# Autodesk Inventor assembly: TopOfRobot
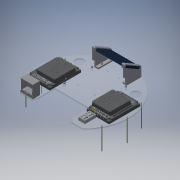
[picture p0: Inventor's stored thumbnail of the model, 180x180]
Saved by Autodesk Inventor 2019 (Build 230136000, 136)
## iProperties
Created: 2019-10-01
Part Number: TopOfRobot
Document SubType Name: Assembly
Designer: james
Author: james
## Documents named in this file (10)
- F:\JimsDesign\Jims2020FTC\TopOfRobot.iam
- F:\JimsDesign\Jims2020FTC\TopPlate.ipt
- F:\JimsDesign\Library\RevRobotics\REV-31-1153.ipt
- F:\JimsDesign\Jims2020FTC\CameraMount v4.ipt
- F:\JimsDesign\Jims2020FTC\SidePeg.ipt
- F:\JimsDesign\Jims2020FTC\CurrentMonitorBlock.ipt
- F:\JimsDesign\Jims2020FTC\PhoneStandLeft.ipt
- F:\JimsDesign\Jims2020FTC\PhoneStandRight.ipt
- F:\JimsDesign\Jims2020FTC\Phone.ipt
- F:\JimsDesign\Library\McMaster\SocketScrews\91251A194_BLACK-OXIDE ALLOY STEEL SOCKET HEAD CAP SCREW.ipt
## Components (23 placed, 9 different names)
1. TopPlate:1 — Mate:1, Mate:2, Mate:3, Mate:4, Mate:5, Mate:6, Mate:7, Mate:8, Mate:9, Mate:10, Mate:11, Mate:12, Flush:1, Flush:2, Flush:3, Mate:13, Mate:14, Mate:15, Flush:4, Flush:5, Flush:6, Mate:16, Mate:17, Mate:18, Mate:19, Mate:20, Mate:21, Mate:23, Mate:24, Mate:27, Mate:28, Mate:29, Mate:30, Mate:31, Mate:32, Mate:33, Mate:34, Mate:35
2. REV-31-1153:1 — Mate:1, Mate:3, Mate:4
3. REV-31-1153:2 — Mate:2, Mate:5, Mate:6
4. CameraMount v4:1 — Mate:7, Mate:8, Mate:9
5. SidePeg:1 — Mate:15, Flush:4
6. SidePeg:2 — Mate:14, Flush:5
7. SidePeg:3 — Mate:13, Flush:6
8. SidePeg:4 — Mate:12, Flush:1
9. SidePeg:5 — Mate:11, Flush:2
10. SidePeg:6 — Mate:10, Flush:3
11. CurrentMonitorBlock:1 — Mate:17, Mate:20, Mate:21
12. CurrentMonitorBlock:2 — Mate:16, Mate:18, Mate:19
13. PhoneStandLeft:1 — Flush:7, Flush:8, Mate:27, Mate:36, Mate:37, Mate:38, Mate:39, Mate:40, Mate:41, Flush:9
14. PhoneStandRight:1 — Flush:7, Flush:8, Mate:23, Mate:24, Mate:25, Mate:42, Mate:43, Mate:44
15. Phone:1 — Mate:25, Mate:44, Flush:9
16. 91251A194_BLACK-OXIDE ALLOY STEEL SOCKET HEAD CAP SCREW:1 — Mate:28, Mate:32
17. 91251A194_BLACK-OXIDE ALLOY STEEL SOCKET HEAD CAP SCREW:2 — Mate:29, Mate:34
18. 91251A194_BLACK-OXIDE ALLOY STEEL SOCKET HEAD CAP SCREW:3 — Mate:31, Mate:35
19. 91251A194_BLACK-OXIDE ALLOY STEEL SOCKET HEAD CAP SCREW:4 — Mate:30, Mate:33
20. 91251A194_BLACK-OXIDE ALLOY STEEL SOCKET HEAD CAP SCREW:5 — Mate:36, Mate:43
21. 91251A194_BLACK-OXIDE ALLOY STEEL SOCKET HEAD CAP SCREW:6 — Mate:37, Mate:42
22. 91251A194_BLACK-OXIDE ALLOY STEEL SOCKET HEAD CAP SCREW:7 — Mate:38, Mate:41
23. 91251A194_BLACK-OXIDE ALLOY STEEL SOCKET HEAD CAP SCREW:8 — Mate:39, Mate:40
## Relationships (51: Mate 42, Flush 9)
- Mate:1: TopPlate:1 ↔ REV-31-1153:1
- Mate:2: TopPlate:1 ↔ REV-31-1153:2
- Mate:3: TopPlate:1 ↔ REV-31-1153:1
- Mate:4: TopPlate:1 ↔ REV-31-1153:1
- Mate:5: TopPlate:1 ↔ REV-31-1153:2
- Mate:6: TopPlate:1 ↔ REV-31-1153:2
- Mate:7: TopPlate:1 ↔ CameraMount v4:1
- Mate:8: TopPlate:1 ↔ CameraMount v4:1
- Mate:9: TopPlate:1 ↔ CameraMount v4:1
- Mate:10: TopPlate:1 ↔ SidePeg:6
- Mate:11: TopPlate:1 ↔ SidePeg:5
- Mate:12: TopPlate:1 ↔ SidePeg:4
- Flush:1: TopPlate:1 ↔ SidePeg:4
- Flush:2: TopPlate:1 ↔ SidePeg:5
- Flush:3: TopPlate:1 ↔ SidePeg:6
- Mate:13: TopPlate:1 ↔ SidePeg:3
- Mate:14: TopPlate:1 ↔ SidePeg:2
- Mate:15: TopPlate:1 ↔ SidePeg:1
- Flush:4: TopPlate:1 ↔ SidePeg:1
- Flush:5: TopPlate:1 ↔ SidePeg:2
- Flush:6: TopPlate:1 ↔ SidePeg:3
- Mate:16: TopPlate:1 ↔ CurrentMonitorBlock:2
- Mate:17: TopPlate:1 ↔ CurrentMonitorBlock:1
- Mate:18: TopPlate:1 ↔ CurrentMonitorBlock:2
- Mate:19: TopPlate:1 ↔ CurrentMonitorBlock:2
- Mate:20: TopPlate:1 ↔ CurrentMonitorBlock:1
- Mate:21: TopPlate:1 ↔ CurrentMonitorBlock:1
- Flush:7: PhoneStandLeft:1 ↔ PhoneStandRight:1
- Flush:8: PhoneStandLeft:1 ↔ PhoneStandRight:1
- Mate:23: TopPlate:1 ↔ PhoneStandRight:1
- Mate:24: TopPlate:1 ↔ PhoneStandRight:1
- Mate:25: PhoneStandRight:1 ↔ Phone:1
- Mate:27: TopPlate:1 ↔ PhoneStandLeft:1
- Mate:28: TopPlate:1 ↔ 91251A194_BLACK-OXIDE ALLOY STEEL SOCKET HEAD CAP SCREW:1
- Mate:29: TopPlate:1 ↔ 91251A194_BLACK-OXIDE ALLOY STEEL SOCKET HEAD CAP SCREW:2
- Mate:30: TopPlate:1 ↔ 91251A194_BLACK-OXIDE ALLOY STEEL SOCKET HEAD CAP SCREW:4
- Mate:31: TopPlate:1 ↔ 91251A194_BLACK-OXIDE ALLOY STEEL SOCKET HEAD CAP SCREW:3
- Mate:32: TopPlate:1 ↔ 91251A194_BLACK-OXIDE ALLOY STEEL SOCKET HEAD CAP SCREW:1
- Mate:33: TopPlate:1 ↔ 91251A194_BLACK-OXIDE ALLOY STEEL SOCKET HEAD CAP SCREW:4
- Mate:34: TopPlate:1 ↔ 91251A194_BLACK-OXIDE ALLOY STEEL SOCKET HEAD CAP SCREW:2
- Mate:35: TopPlate:1 ↔ 91251A194_BLACK-OXIDE ALLOY STEEL SOCKET HEAD CAP SCREW:3
- Mate:36: PhoneStandLeft:1 ↔ 91251A194_BLACK-OXIDE ALLOY STEEL SOCKET HEAD CAP SCREW:5
- Mate:37: PhoneStandLeft:1 ↔ 91251A194_BLACK-OXIDE ALLOY STEEL SOCKET HEAD CAP SCREW:6
- Mate:38: PhoneStandLeft:1 ↔ 91251A194_BLACK-OXIDE ALLOY STEEL SOCKET HEAD CAP SCREW:7
- Mate:39: PhoneStandLeft:1 ↔ 91251A194_BLACK-OXIDE ALLOY STEEL SOCKET HEAD CAP SCREW:8
- Mate:40: PhoneStandLeft:1 ↔ 91251A194_BLACK-OXIDE ALLOY STEEL SOCKET HEAD CAP SCREW:8
- Mate:41: PhoneStandLeft:1 ↔ 91251A194_BLACK-OXIDE ALLOY STEEL SOCKET HEAD CAP SCREW:7
- Mate:42: PhoneStandRight:1 ↔ 91251A194_BLACK-OXIDE ALLOY STEEL SOCKET HEAD CAP SCREW:6
- Mate:43: PhoneStandRight:1 ↔ 91251A194_BLACK-OXIDE ALLOY STEEL SOCKET HEAD CAP SCREW:5
- Mate:44: PhoneStandRight:1 ↔ Phone:1
- Flush:9: PhoneStandLeft:1 ↔ Phone:1
